# Autodesk Inventor assembly: x_axis
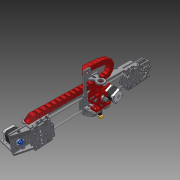
[picture p0: Inventor's stored thumbnail of the model, 180x180]
Saved by Autodesk Inventor 2014 (Build 180170000, 170)
## iProperties
Created: 2013-12-02
Part Number: x_axis
Document SubType Name: Assembly
Designer: buben
Author: buben
## Documents named in this file (14)
- C:\Users\buben\Documents\GitHub\bacon\inventor files\assemblies\x_axis.iam
- C:\Users\buben\Documents\GitHub\bacon\inventor files\assemblies\x_motor.iam
- C:\Users\buben\Documents\GitHub\bacon\inventor files\assemblies\x_iddler.iam
- C:\Users\buben\Documents\GitHub\bacon\inventor files\assemblies\x_carryage.iam
- C:\Users\buben\Documents\GitHub\bacon\inventor files\utils\x_axis_rod.ipt
- C:\Users\buben\Documents\GitHub\bacon\inventor files\printer parts\x_axis_chain_holder.ipt
- C:\Users\buben\Documents\GitHub\bacon\inventor files\utils\x_axis_cable_mount_a.ipt
- C:\Users\buben\Documents\GitHub\bacon\inventor files\utils\washer_m4.ipt
- C:\Users\buben\Documents\Inventor\Content Center Files\R2014\en-US\ISO 7040\ISO 7040 - M4.ipt
- C:\Users\buben\Documents\Inventor\Content Center Files\R2014\en-US\ISO 4762(2)\ISO 4762 - M4 x 30ISO.ipt
- C:\Users\buben\Documents\GitHub\bacon\inventor files\utils\cable_chain_22.ipt
- C:\Users\buben\Documents\GitHub\bacon\inventor files\utils\x_axis_cable_mount_b.ipt
- C:\Users\buben\Documents\GitHub\bacon\inventor files\assemblies\extruder.iam
- C:\Users\buben\Documents\Inventor\Content Center Files\R2014\en-US\ISO 4014(1)\ISO 4014 - M4 x 25DIN EN.ipt
## Components (55 placed, 13 different names)
1. x_motor:1 [sub-assembly] — Mate:1, Mate:2, Mate:3, Flush:1, Flush:2, Mate:7, Tangent:1, Tangent:2, Tangent:3, Tangent:4, Tangent:5, Tangent:6, Mate:11, Mate:12, Mate:23, Mate:25
2. x_iddler:1 [sub-assembly] — Flush:1, Flush:2, Mate:8, Mate:13, Mate:33, Mate:35
3. x_carryage:1 [sub-assembly] — Mate:7, Mate:8, Mate:9, Mate:10, Mate:41, Mate:42, Mate:43, Mate:44, Mate:45, Mate:52, Mate:53
4. x_axis_rod:1 — Tangent:1, Tangent:3, Tangent:5, Mate:10
5. x_axis_rod:2 — Tangent:2, Tangent:4, Tangent:6, Mate:9
6. x_axis_chain_holder:1 — Mate:11, Mate:12, Mate:13, Mate:14, Flush:3, Flush:4, Mate:15, Mate:16, Mate:17, Mate:18, Mate:19, Mate:20, Mate:21, Mate:22
7. x_axis_cable_mount_a:1 — Mate:14, Flush:3, Flush:4, Insert:5, Angle:1
8. CSN 02 1702 B B 4,3:1 — Mate:15, Mate:16, Insert:2
9. CSN 02 1702 B B 4,3:2 — Mate:17, Mate:18, Insert:1
10. CSN 02 1702 B B 4,3:3 — Mate:23, Mate:27, Mate:28
11. CSN 02 1702 B B 4,3:4 — Mate:25, Mate:30, Mate:31
12. CSN 02 1702 B B 4,3:5 — Mate:19, Mate:20, Insert:3
13. CSN 02 1702 B B 4,3:6 — Mate:35, Mate:36, Mate:39
14. CSN 02 1702 B B 4,3:7 — Mate:21, Mate:22, Insert:4
15. CSN 02 1702 B B 4,3:8 — Mate:33, Mate:34, Mate:37
16. DIN EN ISO 7040 M4:1 — Mate:31, Mate:32
17. DIN EN ISO 7040 M4:2 — Mate:39, Mate:40
18. DIN EN ISO 7040 M4:3 — Mate:37, Mate:38
19. DIN EN ISO 7040 M4:4 — Mate:27, Mate:29
20. ISO 4762 M4 x 30:1 — Insert:3, Mate:36, Mate:40
21. ISO 4762 M4 x 30:2 — Insert:4, Mate:34, Mate:38
22. ISO 4762 M4 x 30:3 — Insert:2, Mate:28, Mate:29
23. ISO 4762 M4 x 30:4 — Insert:1, Mate:30, Mate:32
24. cable_chain_22:1 — Insert:5, Angle:1, Insert:6, Angle:2
25. cable_chain_22:2 — Insert:6, Angle:2, Insert:7, Angle:3
26. cable_chain_22:3 — Insert:7, Angle:3, Insert:10, Angle:6
27. cable_chain_22:4 — Insert:10, Angle:6
28. cable_chain_22:5
29. cable_chain_22:6 — Insert:16, Angle:12
30. cable_chain_22:7 — Insert:16, Angle:12
31. cable_chain_22:8
32. cable_chain_22:9
33. cable_chain_22:10
34. cable_chain_22:11
35. cable_chain_22:12 — Insert:28, Angle:24
36. cable_chain_22:13 — Insert:28, Angle:24
37. cable_chain_22:14
38. cable_chain_22:15
39. cable_chain_22:16
40. cable_chain_22:17
41. cable_chain_22:18
42. cable_chain_22:19
43. cable_chain_22:20
44. cable_chain_22:21
45. cable_chain_22:22
46. cable_chain_22:23
47. cable_chain_22:24 — Insert:29, Angle:25
48. x_axis_cable_mount_b:1 — Insert:29, Angle:25, Mate:41, Mate:42
49. extruder:1 [sub-assembly] — Mate:43, Mate:44, Mate:45, Mate:46, Mate:47, Mate:48, Mate:49, Mate:50, Mate:51
50. DIN EN 24014 M4 x 25:1 — Mate:46, Mate:47, Mate:48, Mate:55, Mate:59
51. DIN EN 24014 M4 x 25:2 — Mate:49, Mate:50, Mate:51, Mate:54, Mate:57
52. CSN 02 1702 B B 4,3:9 — Mate:53, Mate:55, Mate:58
53. CSN 02 1702 B B 4,3:10 — Mate:52, Mate:54, Mate:56
54. DIN EN ISO 7040 M4:5 — Mate:58, Mate:59
55. DIN EN ISO 7040 M4:6 — Mate:56, Mate:57
## Relationships (118: Mate 54, Insert 29, Angle 25, Tangent 6, Flush 4)
- Mate:1: x_motor:1
- Mate:2: x_motor:1
- Mate:3: x_motor:1
- Flush:1: x_motor:1 ↔ x_iddler:1
- Flush:2: x_motor:1 ↔ x_iddler:1
- Mate:7: x_motor:1 ↔ x_carryage:1
- Mate:8: x_iddler:1 ↔ x_carryage:1
- Tangent:1: x_motor:1 ↔ x_axis_rod:1
- Tangent:2: x_motor:1 ↔ x_axis_rod:2
- Tangent:3: x_motor:1 ↔ x_axis_rod:1
- Tangent:4: x_motor:1 ↔ x_axis_rod:2
- Tangent:5: x_motor:1 ↔ x_axis_rod:1
- Tangent:6: x_motor:1 ↔ x_axis_rod:2
- Mate:9: x_carryage:1 ↔ x_axis_rod:2
- Mate:10: x_carryage:1 ↔ x_axis_rod:1
- Mate:11: x_motor:1 ↔ x_axis_chain_holder:1
- Mate:12: x_motor:1 ↔ x_axis_chain_holder:1
- Mate:13: x_iddler:1 ↔ x_axis_chain_holder:1
- Mate:14: x_axis_chain_holder:1 ↔ x_axis_cable_mount_a:1
- Flush:3 (1 mm): x_axis_chain_holder:1 ↔ x_axis_cable_mount_a:1
- Flush:4 (5 mm): x_axis_chain_holder:1 ↔ x_axis_cable_mount_a:1
- Mate:15: x_axis_chain_holder:1 ↔ CSN 02 1702 B B 4,3:1
- Mate:16: x_axis_chain_holder:1 ↔ CSN 02 1702 B B 4,3:1
- Mate:17: x_axis_chain_holder:1 ↔ CSN 02 1702 B B 4,3:2
- Mate:18: x_axis_chain_holder:1 ↔ CSN 02 1702 B B 4,3:2
- Mate:19: x_axis_chain_holder:1 ↔ CSN 02 1702 B B 4,3:5
- Mate:20: x_axis_chain_holder:1 ↔ CSN 02 1702 B B 4,3:5
- Mate:21: x_axis_chain_holder:1 ↔ CSN 02 1702 B B 4,3:7
- Mate:22: x_axis_chain_holder:1 ↔ CSN 02 1702 B B 4,3:7
- Mate:23: x_motor:1 ↔ CSN 02 1702 B B 4,3:3
- Mate:25: x_motor:1 ↔ CSN 02 1702 B B 4,3:4
- Mate:27: CSN 02 1702 B B 4,3:3 ↔ DIN EN ISO 7040 M4:4
- Insert:1: CSN 02 1702 B B 4,3:2 ↔ ISO 4762 M4 x 30:4
- Insert:2: CSN 02 1702 B B 4,3:1 ↔ ISO 4762 M4 x 30:3
- Mate:28: CSN 02 1702 B B 4,3:3 ↔ ISO 4762 M4 x 30:3
- Mate:29: DIN EN ISO 7040 M4:4 ↔ ISO 4762 M4 x 30:3
- Mate:30: CSN 02 1702 B B 4,3:4 ↔ ISO 4762 M4 x 30:4
- Mate:31: CSN 02 1702 B B 4,3:4 ↔ DIN EN ISO 7040 M4:1
- Mate:32: DIN EN ISO 7040 M4:1 ↔ ISO 4762 M4 x 30:4
- Insert:3: CSN 02 1702 B B 4,3:5 ↔ ISO 4762 M4 x 30:1
- Insert:4: CSN 02 1702 B B 4,3:7 ↔ ISO 4762 M4 x 30:2
- Mate:33: x_iddler:1 ↔ CSN 02 1702 B B 4,3:8
- Mate:34: CSN 02 1702 B B 4,3:8 ↔ ISO 4762 M4 x 30:2
- Mate:35: x_iddler:1 ↔ CSN 02 1702 B B 4,3:6
- Mate:36: CSN 02 1702 B B 4,3:6 ↔ ISO 4762 M4 x 30:1
- Mate:37: CSN 02 1702 B B 4,3:8 ↔ DIN EN ISO 7040 M4:3
- Mate:38: DIN EN ISO 7040 M4:3 ↔ ISO 4762 M4 x 30:2
- Mate:39: CSN 02 1702 B B 4,3:6 ↔ DIN EN ISO 7040 M4:2
- Mate:40: DIN EN ISO 7040 M4:2 ↔ ISO 4762 M4 x 30:1
- Insert:5: x_axis_cable_mount_a:1 ↔ cable_chain_22:1
- Angle:1 (0 deg): x_axis_cable_mount_a:1 ↔ cable_chain_22:1
- Insert:6: cable_chain_22:1 ↔ cable_chain_22:2
- Angle:2 (0 deg): cable_chain_22:1 ↔ cable_chain_22:2
- Insert:7: cable_chain_22:2 ↔ cable_chain_22:3
- Angle:3 (0 deg): cable_chain_22:2 ↔ cable_chain_22:3
- [Insert]: cable_chain_22:4 ↔ cable_chain_22:5
- [Angle] (0 deg): cable_chain_22:4 ↔ cable_chain_22:5
- [Insert]: cable_chain_22:5 ↔ cable_chain_22:6
- [Angle] (0 deg): cable_chain_22:5 ↔ cable_chain_22:6
- Insert:10: cable_chain_22:3 ↔ cable_chain_22:4
- Angle:6 (0 deg): cable_chain_22:3 ↔ cable_chain_22:4
- [Insert]: cable_chain_22:7 ↔ cable_chain_22:8
- [Angle] (0 deg): cable_chain_22:7 ↔ cable_chain_22:8
- [Insert]: cable_chain_22:8 ↔ cable_chain_22:9
- [Angle] (0 deg): cable_chain_22:8 ↔ cable_chain_22:9
- [Insert]: cable_chain_22:10 ↔ cable_chain_22:11
- [Angle] (0 deg): cable_chain_22:10 ↔ cable_chain_22:11
- [Insert]: cable_chain_22:11 ↔ cable_chain_22:12
- [Angle] (0 deg): cable_chain_22:11 ↔ cable_chain_22:12
- [Insert]: cable_chain_22:9 ↔ cable_chain_22:10
- [Angle] (0 deg): cable_chain_22:9 ↔ cable_chain_22:10
- Insert:16: cable_chain_22:6 ↔ cable_chain_22:7
- Angle:12 (0 deg): cable_chain_22:6 ↔ cable_chain_22:7
- [Insert]: cable_chain_22:13 ↔ cable_chain_22:14
- [Angle] (0 deg): cable_chain_22:13 ↔ cable_chain_22:14
- [Insert]: cable_chain_22:14 ↔ cable_chain_22:15
- [Angle] (0 deg): cable_chain_22:14 ↔ cable_chain_22:15
- [Insert]: cable_chain_22:16 ↔ cable_chain_22:17
- [Angle] (0 deg): cable_chain_22:16 ↔ cable_chain_22:17
- [Insert]: cable_chain_22:17 ↔ cable_chain_22:18
- [Angle] (0 deg): cable_chain_22:17 ↔ cable_chain_22:18
- [Insert]: cable_chain_22:15 ↔ cable_chain_22:16
- [Angle] (0 deg): cable_chain_22:15 ↔ cable_chain_22:16
- [Insert]: cable_chain_22:19 ↔ cable_chain_22:20
- [Angle] (0 deg): cable_chain_22:19 ↔ cable_chain_22:20
- [Insert]: cable_chain_22:20 ↔ cable_chain_22:21
- [Angle] (0 deg): cable_chain_22:20 ↔ cable_chain_22:21
- [Insert]: cable_chain_22:22 ↔ cable_chain_22:23
- [Angle] (0 deg): cable_chain_22:22 ↔ cable_chain_22:23
- [Insert]: cable_chain_22:23 ↔ cable_chain_22:24
- [Angle] (0 deg): cable_chain_22:23 ↔ cable_chain_22:24
- [Insert]: cable_chain_22:21 ↔ cable_chain_22:22
- [Angle] (0 deg): cable_chain_22:21 ↔ cable_chain_22:22
- [Insert]: cable_chain_22:18 ↔ cable_chain_22:19
- [Angle] (0 deg): cable_chain_22:18 ↔ cable_chain_22:19
- Insert:28: cable_chain_22:12 ↔ cable_chain_22:13
- Angle:24 (0 deg): cable_chain_22:12 ↔ cable_chain_22:13
- Insert:29: cable_chain_22:24 ↔ x_axis_cable_mount_b:1
- Angle:25 (0 deg): cable_chain_22:24 ↔ x_axis_cable_mount_b:1
- Mate:41: x_carryage:1 ↔ x_axis_cable_mount_b:1
- Mate:42: x_carryage:1 ↔ x_axis_cable_mount_b:1
- Mate:43: x_carryage:1 ↔ extruder:1
- Mate:44: x_carryage:1 ↔ extruder:1
- Mate:45: x_carryage:1 ↔ extruder:1
- Mate:46: extruder:1 ↔ DIN EN 24014 M4 x 25:1
- Mate:47: extruder:1 ↔ DIN EN 24014 M4 x 25:1
- Mate:48: extruder:1 ↔ DIN EN 24014 M4 x 25:1
- Mate:49: extruder:1 ↔ DIN EN 24014 M4 x 25:2
- Mate:50: extruder:1 ↔ DIN EN 24014 M4 x 25:2
- Mate:51: extruder:1 ↔ DIN EN 24014 M4 x 25:2
- Mate:52: x_carryage:1 ↔ CSN 02 1702 B B 4,3:10
- Mate:53: x_carryage:1 ↔ CSN 02 1702 B B 4,3:9
- Mate:54: DIN EN 24014 M4 x 25:2 ↔ CSN 02 1702 B B 4,3:10
- Mate:55: DIN EN 24014 M4 x 25:1 ↔ CSN 02 1702 B B 4,3:9
- Mate:56: CSN 02 1702 B B 4,3:10 ↔ DIN EN ISO 7040 M4:6
- Mate:57: DIN EN 24014 M4 x 25:2 ↔ DIN EN ISO 7040 M4:6
- Mate:58: CSN 02 1702 B B 4,3:9 ↔ DIN EN ISO 7040 M4:5
- Mate:59: DIN EN 24014 M4 x 25:1 ↔ DIN EN ISO 7040 M4:5
## Named parameters: d83_d80 = 0 deg, d84_d81 = 36 deg, d85_d82 = 0 deg, d86_d76 = 0 deg, d87_d77 = 36 deg, d88_d78 = 0 deg, d89_d79 = 0 mm, d90_d75 = 0 mm, d95_d80 = 0 deg, d96_d81 = 36 deg, d97_d82 = 0 deg, d98_d83_d80 = 0 deg, d99_d84_d81 = 36 deg, d100_d85_d82 = 0 deg, d101_d86_d76 = 0 deg, d102_d87_d77 = 36 deg, d103_d88_d78 = 0 deg, d104_d89_d79 = 0 mm, d105_d90_d75 = 0 mm, d106_d91 = 0 mm, d107_d92 = 0 deg, d108_d93 = 36 deg, d109_d94 = 0 deg, d110_d76 = 0 deg, d111_d77 = 36 deg, d112_d78 = 0 deg, d113_d79 = 0 mm, d114_d75 = 0 mm, d119_d115 = 0 mm, d120_d116 = 0 deg, d121_d117 = 36 deg, d122_d118 = 0 deg, d123_d80 = 0 deg, d124_d81 = 36 deg, d125_d82 = 0 deg, d126_d83_d80 = 0 deg, d127_d84_d81 = 36 deg, d128_d85_d82 = 0 deg, d129_d86_d76 = 0 deg, d130_d87_d77 = 36 deg, d131_d88_d78 = 0 deg, d132_d89_d79 = 0 mm, d133_d90_d75 = 0 mm, d134_d91 = 0 mm, d135_d92 = 0 deg, d136_d93 = 36 deg, d137_d94 = 0 deg, d138_d95_d80 = 0 deg, d139_d96_d81 = 36 deg, d140_d97_d82 = 0 deg, d141_d98_d83_d80 = 0 deg, d142_d99_d84_d81 = 36 deg, d143_d100_d85_d82 = 0 deg, d144_d101_d86_d76 = 0 deg, d145_d102_d87_d77 = 36 deg, d146_d103_d88_d78 = 0 deg, d147_d104_d89_d79 = 0 mm, d148_d105_d90_d75 = 0 mm, d149_d106_d91 = 0 mm, d150_d107_d92 = 0 deg, d151_d108_d93 = 36 deg, d152_d109_d94 = 0 deg, d153_d110_d76 = 0 deg, d154_d111_d77 = 36 deg, d155_d112_d78 = 0 deg, d156_d113_d79 = 0 mm, d157_d114_d75 = 0 mm, d158_d76 = 0 deg, d159_d77 = 36 deg, d160_d78 = 0 deg, d161_d79 = 0 mm, d162_d75 = 0 mm
